# Autodesk Inventor assembly: transistor
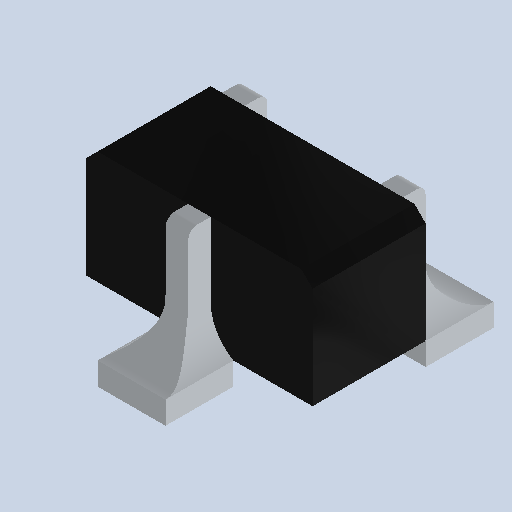
[picture p0: Inventor's stored thumbnail of the model, 512x512]
Saved by Autodesk Inventor 2025 (Build 290162000, 162)
## iProperties
Created: 2025-09-09
Part Number: transistor
Document SubType Name: Assembly
Designer: jirne
Author: jirne
## Documents named in this file (3)
- C:\Users\jirne\JVR11\hardware\library\3D\DCJ11\transistor\transistor.iam
- C:\Users\jirne\JVR11\hardware\library\3D\DCJ11\transistor\connection.ipt
- C:\Users\jirne\JVR11\hardware\library\3D\DCJ11\transistor\body.ipt
## Components (2 placed, 2 different names)
1. connection:1 — Mate:1, Flush:1, Flush:2
2. body:1 — Mate:1, Flush:1, Flush:2
## Relationships (3: Flush 2, Mate 1)
- Mate:1: connection:1 ↔ body:1
- Flush:1: connection:1 ↔ body:1
- Flush:2: connection:1 ↔ body:1
